# Autodesk Inventor assembly: Podstawa(zespol)
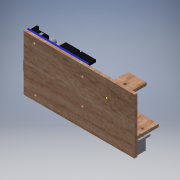
[picture p0: Inventor's stored thumbnail of the model, 180x180]
Saved by Autodesk Inventor 2017 (Build 210142000, 142)
## iProperties
Part Number: Podstawa(zespol)
Material: Ogólny
Document SubType Name: Assembly
Designer: Damian
Author: Damian
## Documents named in this file (4)
- C:\Users\Damian\Documents\Inventor\Nowe\2.0\Podstawa(zespol).iam
- C:\Users\Damian\Documents\Inventor\Nowe\2.0\podstawa.ipt
- C:\Users\Damian\Documents\Inventor\Nowe\2.0\towerpro.ipt
- C:\Users\Damian\Documents\Inventor\Nowe\2.0\Arduino Uno\arduino uno.iam
## Components (3 placed, 3 different names)
1. podstawa:1 — Sztywne:1
2. towerpro:1 — Sztywne:1
3. arduino uno:1 [sub-assembly]
## Relationships (1: WeldJoint 1)
- Sztywne:1 [WeldJoint] (-1 mm): podstawa:1 ↔ towerpro:1
